# Autodesk Inventor assembly: Funnel Wheel Clamp V3
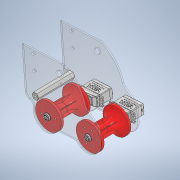
[picture p0: Inventor's stored thumbnail of the model, 180x180]
Saved by Autodesk Inventor 2022 (Build 260153000, 153)
## iProperties
Created: 2022-09-17
Part Number: Funnel Wheel Clamp V3
Document SubType Name: Assembly
Designer: matt
Author: matt
## Documents named in this file (10)
- C:\Users\matt\Documents\Inventor\FTC\2022-23 FTC\Intake\Funnel Wheel Clamp V3.iam
- C:\Users\matt\Documents\Inventor\FTC\2022-23 FTC\Wheels\Custom Intake Wheel_MIR.ipt
- C:\Users\matt\Documents\Inventor\FTC\2022-23 FTC\FTC Robot Parts\Structural\8mm Bearing with Hex Insert_MIR.iam
- C:\Users\matt\Documents\Inventor\FTC\2022-23 FTC\FTC Robot Parts\Servos\REV-41-1097 (1)_MIR.ipt
- C:\Users\matt\Documents\Inventor\FTC\2022-23 FTC\FTC Robot Parts\Shafts\5mm hex shaft_MIR.ipt
- C:\Users\matt\Documents\Inventor\FTC\2022-23 FTC\FTC Robot Parts\Servos\Servo Horn_MIR.ipt
- C:\Users\matt\Documents\Inventor\FTC\2022-23 FTC\Fasteners\M3 x 8 Button Head.ipt
- C:\Users\matt\Documents\Inventor\FTC\2022-23 FTC\Intake\Intake Sides V4_servo.ipt
- C:\Users\matt\Documents\Inventor\FTC\2022-23 FTC\Intake\Intake Sides V4_bearing.ipt
- C:\Users\matt\Documents\Inventor\FTC\2022-23 FTC\FTC Robot Parts\Shafts\spacers.ipt
## Components (22 placed, 9 different names)
1. Custom Intake Wheel_MIR:1 — Mate:32, Flush:2, Mate:12, Mate:74, Mate:30, Mate:84, Angle:1, Mate:22, Mate:23, Mate:31, Mate:61, Angle:2
2. Custom Intake Wheel_MIR:2 — Mate:78, Mate:22, Mate:23, Mate:29, Mate:32, Mate:34, Mate:61
3. Custom Intake Wheel_MIR:3 — Mate:11, Mate:8, Mate:92, Mate:79, Mate:60, Mate:64, Mate:65, Mate:66
4. Custom Intake Wheel_MIR:4 — Flush:2, Mate:12, Mate:11, Mate:8, Mate:73, Mate:72, Mate:30, Mate:60, Angle:2
5. 8mm Bearing with Hex Insert_MIR:1 [sub-assembly] — Mate:74, Mate:30, Flush:6, Mate:55, Mate:62
6. 8mm Bearing with Hex Insert_MIR:2 [sub-assembly] — Mate:73, Mate:72, Flush:5, Mate:51, Mate:54, Mate:63
7. REV-41-1097 (1)_MIR:1 — Mate:81, Mate:80, Mate:46, Mate:47
8. REV-41-1097 (1)_MIR:2 — Mate:28, Mate:45, Mate:48, Mate:49, Mate:50
9. 5mm hex shaft_MIR:1 — Flush:5, Mate:30, Mate:54, Angle:3
10. 5mm hex shaft_MIR:2 — Flush:6, Mate:31, Mate:55, Angle:3
11. Intake Sides V4_servo:1 — Mate:45, Mate:46, Mate:47, Mate:48, Mate:49, Mate:57
12. Servo Horn_MIR:1 — Mate:78, Mate:28, Mate:29, Mate:32, Mate:33, Mate:35, Mate:36, Mate:37, Mate:38, Mate:39, Mate:50
13. Servo Horn_MIR:2 — Mate:92, Mate:81, Mate:80, Mate:79
14. M3 x 8 Button Head:1 — Flush:6, Mate:38
15. M3 x 8 Button Head:2 — Flush:6, Flush:7, Mate:39
16. M3 x 8 Button Head:3 — Flush:7, Flush:8, Mate:37
17. M3 x 8 Button Head:4 — Flush:8, Flush:9, Mate:36
18. M3 x 8 Button Head:5 — Flush:9, Flush:10, Mate:35
19. M3 x 8 Button Head:6 — Flush:10, Mate:33, Mate:34
20. Intake Sides V4_bearing:1 — Mate:51, Mate:62, Mate:63
21. spacers:2 — Mate:57
22. Custom Intake Wheel_MIR:5 — Mate:64, Mate:65, Mate:66
## Relationships (56: Mate 45, Flush 8, Angle 3)
- Mate:32 (44.45 mm): Custom Intake Wheel_MIR:1
- Flush:2: Custom Intake Wheel_MIR:1 ↔ Custom Intake Wheel_MIR:4
- Mate:12 (88.9 mm): Custom Intake Wheel_MIR:1 ↔ Custom Intake Wheel_MIR:4
- Mate:11: Custom Intake Wheel_MIR:3 ↔ Custom Intake Wheel_MIR:4
- Mate:8: Custom Intake Wheel_MIR:3 ↔ Custom Intake Wheel_MIR:4
- Mate:74: Custom Intake Wheel_MIR:1 ↔ 8mm Bearing with Hex Insert_MIR:1
- Mate:30: Custom Intake Wheel_MIR:1 ↔ 8mm Bearing with Hex Insert_MIR:1
- Mate:73: Custom Intake Wheel_MIR:4 ↔ 8mm Bearing with Hex Insert_MIR:2
- Mate:72: Custom Intake Wheel_MIR:4 ↔ 8mm Bearing with Hex Insert_MIR:2
- Flush:5: 8mm Bearing with Hex Insert_MIR:2 ↔ 5mm hex shaft_MIR:1
- Flush:6: 8mm Bearing with Hex Insert_MIR:1 ↔ 5mm hex shaft_MIR:2
- Mate:78: Custom Intake Wheel_MIR:2 ↔ Servo Horn_MIR:1
- Mate:92: Custom Intake Wheel_MIR:3 ↔ Servo Horn_MIR:2
- Mate:81: REV-41-1097 (1)_MIR:1 ↔ Servo Horn_MIR:2
- Mate:80: REV-41-1097 (1)_MIR:1 ↔ Servo Horn_MIR:2
- Mate:79: Custom Intake Wheel_MIR:3 ↔ Servo Horn_MIR:2
- Mate:84: Custom Intake Wheel_MIR:1
- Angle:1 (0 deg): Custom Intake Wheel_MIR:1
- Mate:22: Custom Intake Wheel_MIR:1 ↔ Custom Intake Wheel_MIR:2
- Mate:23: Custom Intake Wheel_MIR:1 ↔ Custom Intake Wheel_MIR:2
- Mate:28: REV-41-1097 (1)_MIR:2 ↔ Servo Horn_MIR:1
- Mate:29: Custom Intake Wheel_MIR:2 ↔ Servo Horn_MIR:1
- Mate:30: Custom Intake Wheel_MIR:4 ↔ 5mm hex shaft_MIR:1
- Mate:31: Custom Intake Wheel_MIR:1 ↔ 5mm hex shaft_MIR:2
- Mate:32: Custom Intake Wheel_MIR:2 ↔ Servo Horn_MIR:1
- Flush:6: M3 x 8 Button Head:1 ↔ M3 x 8 Button Head:2
- Flush:7: M3 x 8 Button Head:2 ↔ M3 x 8 Button Head:3
- Flush:8: M3 x 8 Button Head:3 ↔ M3 x 8 Button Head:4
- Flush:9: M3 x 8 Button Head:4 ↔ M3 x 8 Button Head:5
- Flush:10: M3 x 8 Button Head:5 ↔ M3 x 8 Button Head:6
- Mate:33: Servo Horn_MIR:1 ↔ M3 x 8 Button Head:6
- Mate:34: Custom Intake Wheel_MIR:2 ↔ M3 x 8 Button Head:6
- Mate:35: Servo Horn_MIR:1 ↔ M3 x 8 Button Head:5
- Mate:36: Servo Horn_MIR:1 ↔ M3 x 8 Button Head:4
- Mate:37: Servo Horn_MIR:1 ↔ M3 x 8 Button Head:3
- Mate:38: Servo Horn_MIR:1 ↔ M3 x 8 Button Head:1
- Mate:39: Servo Horn_MIR:1 ↔ M3 x 8 Button Head:2
- Mate:45: REV-41-1097 (1)_MIR:2 ↔ Intake Sides V4_servo:1
- Mate:46: REV-41-1097 (1)_MIR:1 ↔ Intake Sides V4_servo:1
- Mate:47: REV-41-1097 (1)_MIR:1 ↔ Intake Sides V4_servo:1
- Mate:48: REV-41-1097 (1)_MIR:2 ↔ Intake Sides V4_servo:1
- Mate:49: REV-41-1097 (1)_MIR:2 ↔ Intake Sides V4_servo:1
- Mate:50: REV-41-1097 (1)_MIR:2 ↔ Servo Horn_MIR:1
- Mate:51: 8mm Bearing with Hex Insert_MIR:2 ↔ Intake Sides V4_bearing:1
- Mate:54: 8mm Bearing with Hex Insert_MIR:2 ↔ 5mm hex shaft_MIR:1
- Mate:55: 8mm Bearing with Hex Insert_MIR:1 ↔ 5mm hex shaft_MIR:2
- Mate:57: Intake Sides V4_servo:1 ↔ spacers:2
- Mate:60: Custom Intake Wheel_MIR:3 ↔ Custom Intake Wheel_MIR:4
- Mate:61: Custom Intake Wheel_MIR:1 ↔ Custom Intake Wheel_MIR:2
- Angle:2 (0 deg): Custom Intake Wheel_MIR:1 ↔ Custom Intake Wheel_MIR:4
- Mate:62: 8mm Bearing with Hex Insert_MIR:1 ↔ Intake Sides V4_bearing:1
- Mate:63: 8mm Bearing with Hex Insert_MIR:2 ↔ Intake Sides V4_bearing:1
- Angle:3 (0 deg): 5mm hex shaft_MIR:1 ↔ 5mm hex shaft_MIR:2
- Mate:64: Custom Intake Wheel_MIR:3 ↔ Custom Intake Wheel_MIR:5
- Mate:65: Custom Intake Wheel_MIR:3 ↔ Custom Intake Wheel_MIR:5
- Mate:66: Custom Intake Wheel_MIR:3 ↔ Custom Intake Wheel_MIR:5
